# Autodesk Inventor assembly: motor_mount_sub_assem
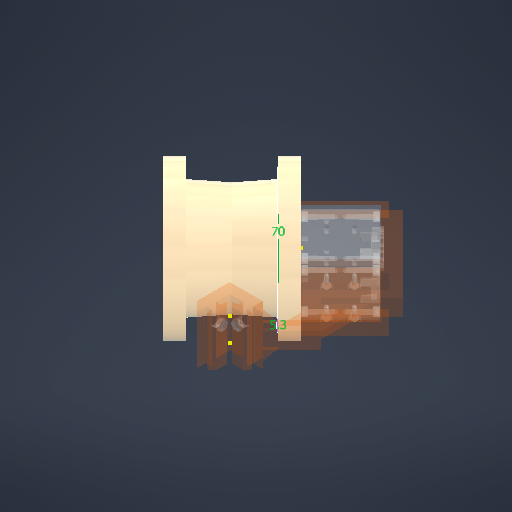
[picture p0: Inventor's stored thumbnail of the model, 512x512]
Saved by Autodesk Inventor 2026.2 (Build 302298010, 298A)
## iProperties
Created: 2026-03-01
Part Number: motor_mount_sub_assem
Document SubType Name: Assembly
Designer: Luke
Author: Luke
## Documents named in this file (5)
- C:\Users\Luke\OneDrive - Heriot-Watt University\Desktop\Robot Mech Sys\GroupProject\CAD\sub_assemblies\motor_mount_sub_assem.iam
- C:\Users\Luke\OneDrive - Heriot-Watt University\Desktop\Robot Mech Sys\GroupProject\CAD\parts\MOTOR_MOUNT_.ipt
- C:\Users\Luke\OneDrive - Heriot-Watt University\Desktop\Robot Mech Sys\GroupProject\CAD\sub_assemblies\motor_spool_sub_assem.iam
- C:\Users\Luke\Documents\Inventor\Content Center Files\R2026\en-US\AS 1427(05)\AS 1427 - M2.5 x 8(5) II.ipt
- C:\Users\Luke\Documents\Inventor\Content Center Files\R2026\en-US\BS EN ISO 7045 H\EN ISO 7045 - M2 x 6 - 4.8 - H(1).ipt
## Components (7 placed, 4 different names)
1. MOTOR_MOUNT_:1 — Mate:1, Mate:2, Mate:3, Mate:8, Mate:9, Mate:10, Mate:11
2. motor_spool_sub_assem:1 [sub-assembly] — Mate:1, Mate:2, Mate:3
3. BS EN ISO 7045 H - Metric M2 x 6 - 4.8 - H:4 — Mate:11
4. AS 1427 H - Metric M2.5 x 8:2
5. BS EN ISO 7045 H - Metric M2 x 6 - 4.8 - H:2 — Mate:10
6. BS EN ISO 7045 H - Metric M2 x 6 - 4.8 - H:1 — Mate:8
7. BS EN ISO 7045 H - Metric M2 x 6 - 4.8 - H:3 — Mate:9
## Relationships (11: Mate 11)
- Mate:1: MOTOR_MOUNT_:1 ↔ motor_spool_sub_assem:1
- Mate:2: MOTOR_MOUNT_:1 ↔ motor_spool_sub_assem:1
- Mate:3: MOTOR_MOUNT_:1 ↔ motor_spool_sub_assem:1
- [Mate]: MOTOR_MOUNT_:1 ↔ BS EN ISO 7045 H - Metric M2 x 6 - 4.8 - H:4
- [Mate]: MOTOR_MOUNT_:1 ↔ BS EN ISO 7045 H - Metric M2 x 6 - 4.8 - H:1
- [Mate]: MOTOR_MOUNT_:1 ↔ BS EN ISO 7045 H - Metric M2 x 6 - 4.8 - H:2
- [Mate]: MOTOR_MOUNT_:1 ↔ BS EN ISO 7045 H - Metric M2 x 6 - 4.8 - H:3
- Mate:8: MOTOR_MOUNT_:1 ↔ BS EN ISO 7045 H - Metric M2 x 6 - 4.8 - H:1
- Mate:9: MOTOR_MOUNT_:1 ↔ BS EN ISO 7045 H - Metric M2 x 6 - 4.8 - H:3
- Mate:10: MOTOR_MOUNT_:1 ↔ BS EN ISO 7045 H - Metric M2 x 6 - 4.8 - H:2
- Mate:11: MOTOR_MOUNT_:1 ↔ BS EN ISO 7045 H - Metric M2 x 6 - 4.8 - H:4
